# Autodesk Inventor assembly: SCHUNK-1401285 AUB Co-act EGP 40 0/12, Fingereinsatz Typ A Co-act EGP-C
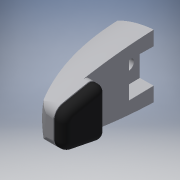
[picture p0: Inventor's stored thumbnail of the model, 180x180]
Saved by Autodesk Inventor 2019 (Build 230136000, 136)
## iProperties
Category: PARTsolutions
Company: SCHUNK
Created: 2022-08-31
Part Number: SCHUNK-1401285 AUB Co-act EGP 40 0/12, Fingereinsatz Typ A Co-act EGP-C
Catalog Web Link: www.cadenas.de
Description: AUB Co-act EGP-Top jaw AUB Co-act EGP
Vendor: SCHUNK
Document SubType Name: Assembly
Designer: psAdmin
Manufacturer: SCHUNK
Mass: 16.0753 g
Surface Area: 67.1782 cm^2
Volume: 16.0753 cm^3
Density: 1 g/cm^3
Title: SCHUNK-1401285 AUB Co-act EGP 40 0/12
Author: Cadenas PARTsolutions
Comments: Top jaw AUB Co-act EGP
PSOL_IDENT_0: {$CADENAS_DATA/23d-libs/schunk/greifsysteme/greifmodule/co_act/co_act_egp_c/aub_co_act_asm_at.prj},2
PSOL_IDENT_1: 84 {VTYP=3D},{STYP=ASSTAB},{NB=SCHUNK-1401285 AUB Co-act EGP 40 0/12, Fingereinsatz Typ A Co-act EGP
PSOL_IDENT_2: -C},{LINA=SCHUNK-1401285 AUB Co-act EGP 40 0/12},{NN=AUB Co-act EGP},{DATE=01.06.2022 15:35:10},{GEO
PSOL_IDENT_3: MDATE=21.12.2021 12:21:13},{VERSION=},{LINEID=30},{WBVAR=AUSWAHLEINSATZ},{WBNUMERIC=}  {NB=SCHUNK-14
PSOL_IDENT_4: 01285 AUB Co-act EGP 40 0/12, Fingereinsatz Typ A Co-act EGP-C},{LINA=SCHUNK-1401285 AUB Co-act EGP
PSOL_IDENT_5: 40 0/12},{KT=DUMMY},{IDNR=1401285},{TYP=AUB Co-act EGP 40 0/12},{ONLINE=Zur Produktseite},{INFOXX=ht
PSOL_IDENT_6: tps://schunk.com/gb_en/gripping-systems/product/65895-0},{AUSWAHLEINSATZ=Fingereinsatz Typ A Co-act
PSOL_IDENT_7: EGP-C},{TYP1=1.000},{PPATH=aub_co_act_asmsbl.prj},{CNSCTN=84662098},{EPIMID=65895}
NB: SCHUNK-1401285 AUB Co-act EGP 40 0/12, Fingereinsatz Typ A Co-act EGP-C
NN: AUB Co-act EGP
NT: Top jaw AUB Co-act EGP
NBSYN: SCHUNK-$IDNR. $TYP., $AUSWAHLEINSATZ.
LINA: SCHUNK-1401285 AUB Co-act EGP 40 0/12
CATALOG: SCHUNK
IDNR: 1401285
TYP: AUB Co-act EGP 40 0/12
ONLINE: To the product page
AUSWAHLEINSATZ: 1352153 - finger insert type A
CNSCTN: 84662098
SUPPLIER: SCHUNK
ARTICLENO: SCHUNK-1401285 AUB Co-act EGP 40 0/12, Fingereinsatz Typ A Co-act EGP-C
BOMINFO: SCHUNK-1401285 AUB Co-act EGP 40 0/12
CREATOR: CADENAS GmbH
## Documents named in this file (4)
- e:\temp\worker_COMMON_2\temp\exporttempdir_4540_36_fj2T2\format_0\SCHUNK-1401285 AUB Co-act EGP 40 0_12, Fingereinsatz Typ A Co-act EGP-C.iam
- e:\temp\worker_COMMON_2\temp\exporttempdir_4540_36_fj2T2\format_0\Dummy SCHUNK-1401285 AUB Co-act EGP 40 0_12, Fingereinsatz Typ A Co-act EGP-C.ipt
- e:\temp\worker_COMMON_2\temp\exporttempdir_4540_36_fj2T2\format_0\SCHUNK-1012602-FIN Co-act EGP 40_12.ipt
- e:\temp\worker_COMMON_2\temp\exporttempdir_4540_36_fj2T2\format_0\SCHUNK-1352153-Fingereinsatz Typ A Co-act EGP-C.ipt
## Components (3 placed, 3 different names)
1. Dummy SCHUNK-1401285 AUB Co-act EGP 40 0_12, Fingereinsatz Typ A Co-act EGP-C:1 — DUMMY_XY@1 <-> AUB_DUMMY_XY@2, DUMMY_Z@1 <-> AUB_DUMMY_Z@2, DUMMY_YZ@1 <-> AUB_DUMMY_YZ@2
2. SCHUNK-1012602-FIN Co-act EGP 40_12:1 — DUMMY_XY@1 <-> AUB_DUMMY_XY@2, DUMMY_Z@1 <-> AUB_DUMMY_Z@2, DUMMY_YZ@1 <-> AUB_DUMMY_YZ@2, AUB_XY@2 <-> EIS_XY@3, AUB_Z@2 <-> EIS_Z@3, AUB_YZ@2 <-> EIS_YZ@3
3. SCHUNK-1352153-Fingereinsatz Typ A Co-act EGP-C:1 — AUB_XY@2 <-> EIS_XY@3, AUB_Z@2 <-> EIS_Z@3, AUB_YZ@2 <-> EIS_YZ@3
## Relationships (6: Flush 2, Mate 2, Angle 2)
- DUMMY_XY@1 <-> AUB_DUMMY_XY@2 [Flush]: Dummy SCHUNK-1401285 AUB Co-act EGP 40 0_12, Fingereinsatz Typ A Co-act EGP-C:1 ↔ SCHUNK-1012602-FIN Co-act EGP 40_12:1
- DUMMY_Z@1 <-> AUB_DUMMY_Z@2 [Mate]: Dummy SCHUNK-1401285 AUB Co-act EGP 40 0_12, Fingereinsatz Typ A Co-act EGP-C:1 ↔ SCHUNK-1012602-FIN Co-act EGP 40_12:1
- DUMMY_YZ@1 <-> AUB_DUMMY_YZ@2 [Angle] (0 deg): Dummy SCHUNK-1401285 AUB Co-act EGP 40 0_12, Fingereinsatz Typ A Co-act EGP-C:1 ↔ SCHUNK-1012602-FIN Co-act EGP 40_12:1
- AUB_XY@2 <-> EIS_XY@3 [Flush]: SCHUNK-1012602-FIN Co-act EGP 40_12:1 ↔ SCHUNK-1352153-Fingereinsatz Typ A Co-act EGP-C:1
- AUB_Z@2 <-> EIS_Z@3 [Mate]: SCHUNK-1012602-FIN Co-act EGP 40_12:1 ↔ SCHUNK-1352153-Fingereinsatz Typ A Co-act EGP-C:1
- AUB_YZ@2 <-> EIS_YZ@3 [Angle] (180 deg): SCHUNK-1012602-FIN Co-act EGP 40_12:1 ↔ SCHUNK-1352153-Fingereinsatz Typ A Co-act EGP-C:1
